# Autodesk Inventor assembly: Chassis_04
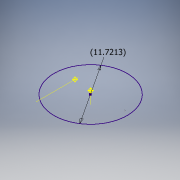
[picture p0: Inventor's stored thumbnail of the model, 180x180]
Saved by Autodesk Inventor 2017 (Build 210142000, 142)
## iProperties
Created: 2017-01-26
Part Number: Chassis_04
Document SubType Name: Assembly
Designer: David Kopala
Author: David Kopala
## Documents named in this file (5)
- Z:\Documents\Drone\Drone\3D Models\Project\Chassis_04\Chassis_04.iam
- Z:\Documents\Drone\Drone\3D Models\Project\Chassis_04\OuterShell.ipt
- Z:\Documents\Drone\Drone\3D Models\Project\Chassis_04\Layer2_Ass.iam
- Z:\Documents\Drone\Drone\3D Models\Project\Chassis_04\Bevel_Ass.iam
- Z:\Documents\Drone\Drone\3D Models\Project\Chassis_04\MotorMount.iam
## Components (4 placed, 4 different names)
1. OuterShell:1 — Insert:1
2. Layer2_Ass:1 [sub-assembly] — Insert:1, Insert:2
3. Bevel_Ass:1 [sub-assembly] — Insert:2
4. MotorMount:1 [sub-assembly]
## Relationships (2: Insert 2)
- Insert:1 (1.5875 mm): OuterShell:1 ↔ Layer2_Ass:1
- Insert:2 (1.5875 mm): Layer2_Ass:1 ↔ Bevel_Ass:1
## Named parameters: IDia = 266.7 mm, Wall = 1.5875 mm, Space = 1.5875 mm, SpWall = 3.175 mm, IBDia = 279.12179 mm, BevOutInDia = 287.59534 mm, BevOutOutDia = 297.72142 mm, BevDriverDia = 23.78518 mm, d1_1 = 6.35 mm, AxelDia = 6.35 mm
